# Autodesk Inventor assembly: Head
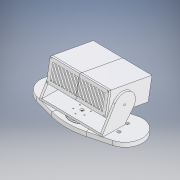
[picture p0: Inventor's stored thumbnail of the model, 180x180]
Saved by Autodesk Inventor 2017 SP1 (Build 210196100, 196)
## iProperties
Created: 2017-06-08
Part Number: Head
Document SubType Name: Assembly
Designer: zallen
Author: zallen
## Documents named in this file (9)
- C:\Users\Zach\Documents\GitHub\tr1\src\Head\Head.iam
- C:\Users\Zach\Documents\GitHub\tr1\src\Head\HA002.ipt
- C:\Users\Zach\Documents\GitHub\tr1\src\Head\HA004.ipt
- C:\Users\Zach\Documents\GitHub\tr1\src\Head\HA005.ipt
- C:\Users\Zach\Documents\GitHub\tr1\src\Head\HA006.ipt
- C:\Users\Zach\Documents\GitHub\tr1\lib\Xbox One Kinect\AS1.iam
- C:\Users\Zach\Documents\GitHub\tr1\src\Head\HA001.ipt
- C:\Users\Zach\Documents\GitHub\tr1\src\Head\HA007.ipt
- C:\Users\Zach\Documents\GitHub\tr1\lib\Strain Wave Gearbox\StrainWaveGearbox.iam
## Components (10 placed, 8 different names)
1. HA001:1 — Mate:24, Mate:25, Mate:35
2. HA002:1 — Mate:1, Mate:9, Mate:26, Mate:27, Mate:28, Mate:29, Mate:30, Mate:42, Mate:43, Mate:44
3. HA004:1 — Mate:7, Mate:21, Mate:39, Mate:40, Mate:41
4. HA005:1 — Mate:7, Mate:13, Mate:17, Mate:19, Mate:20, Mate:21, Mate:24, Mate:25, Mate:33
5. HA006:1 — Mate:13, Mate:32, Mate:34, Flush:1, Mate:35
6. Kinect:1 [sub-assembly] — Mate:17, Mate:19, Mate:20
7. HA007:1 — Mate:26, Mate:27
8. HA007:2 — Mate:28, Mate:29, Mate:30
9. HA006:2 — Mate:32, Mate:33, Mate:34, Flush:1
10. StrainWaveGearbox:1 [sub-assembly] — Mate:39, Mate:40, Mate:41, Mate:42, Mate:43
## Relationships (26: Mate 25, Flush 1)
- Mate:1: HA002:1
- Mate:7: HA004:1 ↔ HA005:1
- Mate:9: HA002:1
- Mate:13: HA005:1 ↔ HA006:1
- Mate:17: HA005:1 ↔ Kinect:1
- Mate:19: HA005:1 ↔ Kinect:1
- Mate:20: HA005:1 ↔ Kinect:1
- Mate:21: HA004:1 ↔ HA005:1
- Mate:24: HA001:1 ↔ HA005:1
- Mate:25: HA001:1 ↔ HA005:1
- Mate:26: HA002:1 ↔ HA007:1
- Mate:27: HA002:1 ↔ HA007:1
- Mate:28: HA002:1 ↔ HA007:2
- Mate:29: HA002:1 ↔ HA007:2
- Mate:30: HA002:1 ↔ HA007:2
- Mate:32: HA006:1 ↔ HA006:2
- Mate:33: HA005:1 ↔ HA006:2
- Mate:34: HA006:1 ↔ HA006:2
- Flush:1: HA006:1 ↔ HA006:2
- Mate:35: HA001:1 ↔ HA006:1
- Mate:39: HA004:1 ↔ StrainWaveGearbox:1
- Mate:40: HA004:1 ↔ StrainWaveGearbox:1
- Mate:41: HA004:1 ↔ StrainWaveGearbox:1
- Mate:42: HA002:1 ↔ StrainWaveGearbox:1
- Mate:43: HA002:1 ↔ StrainWaveGearbox:1
- Mate:44: HA002:1
